# Autodesk Inventor assembly: linear_module_test
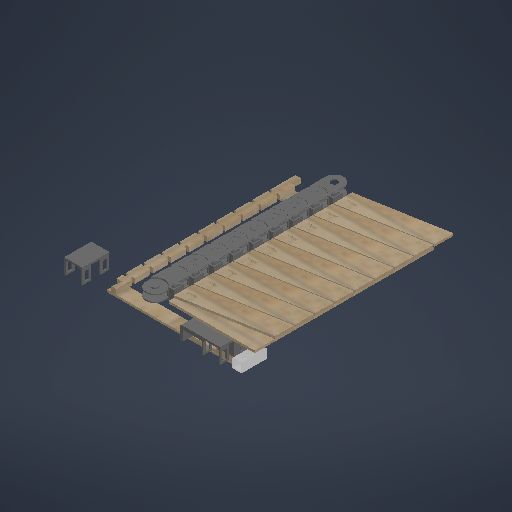
[picture p0: Inventor's stored thumbnail of the model, 512x512]
Saved by Autodesk Inventor 2026.1 (Build 301233020, 233B)
## iProperties
Created: 2025-09-27
Part Number: linear_module_test
Document SubType Name: Assembly
Designer: hibik
Author: hibik
## Documents named in this file (6)
- C:\Users\hibik\Documents\Robomech\conveyer\liniar_module\linear_module_test.iam
- C:\Users\hibik\Documents\Robomech\conveyer\liniar_module\Assy_linear_module.iam
- C:\Users\hibik\Documents\Robomech\conveyer\belt\belt_linear.iam
- C:\Users\hibik\Documents\Robomech\conveyer\connector_module\connetcor_female.ipt
- C:\Users\hibik\Documents\Robomech\conveyer\connector_module\connetcor_female_cover.ipt
- C:\Users\hibik\Documents\Robomech\conveyer\connector_module\position_setter_bar.ipt
## Components (5 placed, 5 different names)
1. Assy_linear_module:1 [sub-assembly] — メイト:1, メイト:2, フラッシュ:1, メイト:3, メイト:4, メイト:5, メイト:6, メイト:7, メイト:8, メイト:9, メイト:10, フラッシュ:2
2. belt_linear:1 [sub-assembly] — メイト:1, メイト:2, フラッシュ:1
3. connetcor_female:1 — メイト:3, メイト:4, メイト:5
4. connetcor_female_cover:1 — メイト:6, メイト:7, メイト:8
5. position_setter_bar:1 — メイト:9, メイト:10, フラッシュ:2
## Relationships (12: Mate 10, Flush 2)
- メイト:1 [Mate]: Assy_linear_module:1 ↔ belt_linear:1
- メイト:2 [Mate]: Assy_linear_module:1 ↔ belt_linear:1
- フラッシュ:1 [Flush] (-11 mm): Assy_linear_module:1 ↔ belt_linear:1
- メイト:3 [Mate] (0.5 mm): Assy_linear_module:1 ↔ connetcor_female:1
- メイト:4 [Mate] (0.6 mm): Assy_linear_module:1 ↔ connetcor_female:1
- メイト:5 [Mate] (0.5 mm): Assy_linear_module:1 ↔ connetcor_female:1
- メイト:6 [Mate] (0.5 mm): Assy_linear_module:1 ↔ connetcor_female_cover:1
- メイト:7 [Mate] (0.5 mm): Assy_linear_module:1 ↔ connetcor_female_cover:1
- メイト:8 [Mate] (0.6 mm): Assy_linear_module:1 ↔ connetcor_female_cover:1
- メイト:9 [Mate] (0.5 mm): Assy_linear_module:1 ↔ position_setter_bar:1
- メイト:10 [Mate] (0.5 mm): Assy_linear_module:1 ↔ position_setter_bar:1
- フラッシュ:2 [Flush]: Assy_linear_module:1 ↔ position_setter_bar:1
